# Autodesk Inventor assembly: Drive
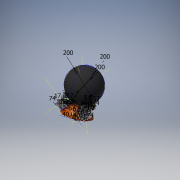
[picture p0: Inventor's stored thumbnail of the model, 180x180]
Saved by Autodesk Inventor 2018.3 (Build 223284000, 284)
## iProperties
Created: 2018-06-30
Part Number: Drive
Material: Generisch
Document SubType Name: Assembly
Designer: JochenAlt
Author: JochenAlt
## Documents named in this file (3)
- D:\Projects\FlowerPot\CAD\Drive.iam
- D:\Projects\FlowerPot\CAD\DriveChain.iam
- D:\Projects\FlowerPot\CAD\Sphere.ipt
## Components (4 placed, 2 different names)
1. Antriebsstrang:1 [sub-assembly] — Passend:1, Passend:2, Fluchtend:1, Fluchtend:2, Passend:3, Passend:4, Passend:6, Passend:7, Passend:9, Passend:10
2. Antriebsstrang:2 [sub-assembly] — Passend:2, Fluchtend:1, Passend:4, Passend:5, Passend:8, Passend:9
3. Antriebsstrang:3 [sub-assembly] — Passend:1, Fluchtend:2, Passend:3, Passend:7, Passend:8
4. Sphere:1 — Passend:5, Passend:10
## Relationships (12: Mate 10, Flush 2)
- Passend:1 [Mate]: Antriebsstrang:1 ↔ Antriebsstrang:3
- Passend:2 [Mate]: Antriebsstrang:1 ↔ Antriebsstrang:2
- Fluchtend:1 [Flush]: Antriebsstrang:1 ↔ Antriebsstrang:2
- Fluchtend:2 [Flush]: Antriebsstrang:1 ↔ Antriebsstrang:3
- Passend:3 [Mate]: Antriebsstrang:1 ↔ Antriebsstrang:3
- Passend:4 [Mate]: Antriebsstrang:1 ↔ Antriebsstrang:2
- Passend:5 [Mate]: Antriebsstrang:2 ↔ Sphere:1
- Passend:6 [Mate]: Antriebsstrang:1
- Passend:7 [Mate]: Antriebsstrang:1 ↔ Antriebsstrang:3
- Passend:8 [Mate]: Antriebsstrang:2 ↔ Antriebsstrang:3
- Passend:9 [Mate]: Antriebsstrang:1 ↔ Antriebsstrang:2
- Passend:10 [Mate]: Antriebsstrang:1 ↔ Sphere:1
